# Autodesk Inventor assembly: am-940a-6-HiGrip-
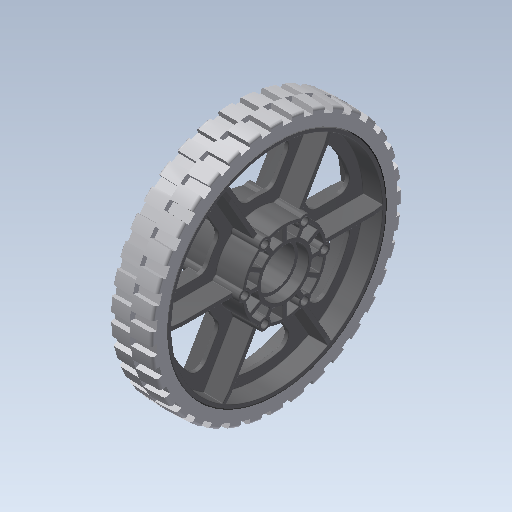
[picture p0: Inventor's stored thumbnail of the model, 512x512]
Saved by Autodesk Inventor 2020 (Build 240168000, 168)
## iProperties
Created: 2014-03-19
Part Number: am-940a-6-HiGrip-
Description: STEP AP214
Document SubType Name: Assembly
Designer: 272834E
Sending System: SolidWorks 2010
Preprocessor: SwSTEP 2.0
Title: 6-HiGrip-am-940aSTEP.STEP
Revision Number: ANY
## Documents named in this file (3)
- C:\Users\lucky\Documents\Inventor\2020DRIVEBASE\6 in HiGrip Wheel\am-940a-6-HiGrip-.iam
- C:\Users\lucky\Documents\Inventor\2020DRIVEBASE\6 in HiGrip Wheel\6 wheel Rev 4.ipt
- C:\Users\lucky\Documents\Inventor\2020DRIVEBASE\6 in HiGrip Wheel\6 wheel tread II.ipt
## Components (2 placed, 2 different names)
1. 6 wheel Rev 4_1 — Mate:1, Flush:1
2. 6 wheel tread II_2 — Mate:1, Flush:1
## Relationships (2: Mate 1, Flush 1)
- Mate:1: 6 wheel Rev 4_1 ↔ 6 wheel tread II_2
- Flush:1: 6 wheel Rev 4_1 ↔ 6 wheel tread II_2
